# Autodesk Inventor assembly: power distribution
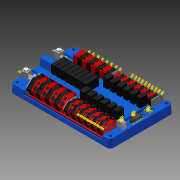
[picture p0: Inventor's stored thumbnail of the model, 180x180]
Saved by Autodesk Inventor 2011 (Build 150239000, 239)
## iProperties
Created: 2010-02-10
Part Number: power distribution
Document SubType Name: Assembly
Designer: a
Author: a
## Documents named in this file (3)
- R:\2012\Inventor\vkop\All-Control-System\power distribution.iam
- R:\2012\Inventor\vkop\All-Control-System\Control System_Diversified_Systems_A003206.ipt
- R:\2012\Inventor\vkop\All-Electrical\Terminal Lug _Burndy_KPA4C.iam
## Components (3 placed, 2 different names)
1. Control System_Diversified_Systems_A003206:1 — Mate:1, Mate:2, Angle:1, Mate:3, Mate:4
2. Terminal Lug _Burndy_KPA4C:1 [sub-assembly] — Mate:1, Mate:2, Angle:1
3. Terminal Lug _Burndy_KPA4C:2 [sub-assembly] — Mate:3, Mate:4
## Relationships (6: Mate 4, Angle 2)
- Mate:1: Control System_Diversified_Systems_A003206:1 ↔ Terminal Lug _Burndy_KPA4C:1
- Mate:2: Control System_Diversified_Systems_A003206:1 ↔ Terminal Lug _Burndy_KPA4C:1
- Angle:1 (0 deg): Control System_Diversified_Systems_A003206:1 ↔ Terminal Lug _Burndy_KPA4C:1
- Mate:3: Control System_Diversified_Systems_A003206:1 ↔ Terminal Lug _Burndy_KPA4C:2
- Mate:4: Control System_Diversified_Systems_A003206:1 ↔ Terminal Lug _Burndy_KPA4C:2
- [Angle] (20 deg): Control System_Diversified_Systems_A003206:1 ↔ Terminal Lug _Burndy_KPA4C:2
